# Autodesk Inventor assembly: Assembly1
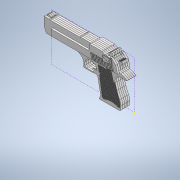
[picture p0: Inventor's stored thumbnail of the model, 180x180]
Saved by Autodesk Inventor 2022 (Build 260153000, 153)
## iProperties
Created: 2022-05-17
Part Number: Assembly1
Document SubType Name: Weldment
Designer: joshn
Weld Material: Welded Aluminum-6061
Author: joshn
## Documents named in this file (9)
- D:\Joshwin Emmanuel\Fab_accad\git_hub\Fab_Work\Wild card\Assembly\Assembly1.iam
- D:\Joshwin Emmanuel\Fab_accad\git_hub\Fab_Work\Wild card\sheetmettaal.ipt
- D:\Joshwin Emmanuel\Fab_accad\git_hub\Fab_Work\Wild card\sheetmettaal_2.ipt
- D:\Joshwin Emmanuel\Fab_accad\git_hub\Fab_Work\Wild card\sheetmettaal_3.ipt
- D:\Joshwin Emmanuel\Fab_accad\git_hub\Fab_Work\Wild card\slider.ipt
- D:\Joshwin Emmanuel\Fab_accad\git_hub\Fab_Work\Wild card\TRIGGER_1.ipt
- D:\Joshwin Emmanuel\Fab_accad\git_hub\Fab_Work\Wild card\TRIGGER_2.ipt
- D:\Joshwin Emmanuel\Fab_accad\git_hub\Fab_Work\Wild card\inner slider.ipt
- D:\Joshwin Emmanuel\Fab_accad\git_hub\Fab_Work\Wild card\FINALcASEING.ipt
## Components (20 placed, 8 different names)
1. sheetmettaal:1 — Mate:1, Mate:2, Mate:3, Mate:4, Flush:1, Flush:2, Mate:7, Flush:6, Flush:12, Flush:22, Flush:32, Mate:34, Mate:35
2. sheetmettaal_2:1 — Mate:4, Flush:1, Flush:2, Flush:3
3. sheetmettaal_3:1 — Flush:3, Mate:5, Flush:4, Flush:5, Flush:8
4. sheetmettaal_2:2 — Mate:5, Flush:4, Flush:5, Mate:8, Mate:9, Mate:11, Flush:11
5. slider:1 — Mate:7, Flush:6, Flush:7, Flush:13
6. slider:2 — Mate:8, Mate:9, Flush:7, Flush:28, Flush:29
7. TRIGGER_1:1 — Flush:8, Flush:10, Mate:17, Flush:25, Flush:26
8. TRIGGER_2:1 — Mate:10, Flush:9, Mate:17, Flush:25, Flush:26
9. TRIGGER_1:2 — Mate:10, Flush:9, Flush:10
10. sheetmettaal:2 — Mate:11, Flush:11, Flush:12, Mate:16, Mate:18
11. inner slider:1 — Flush:13, Flush:14, Mate:12, Flush:15, Mate:13, Flush:17
12. inner slider:2 — Flush:18, Flush:19, Mate:14, Mate:15, Flush:21
13. inner slider:3 — Flush:14, Mate:12, Flush:15, Flush:16
14. inner slider:4 — Flush:16, Mate:13, Flush:17, Mate:15, Flush:20, Flush:21
15. inner slider:5 — Flush:18, Flush:19, Mate:14, Flush:20, Flush:23, Flush:27
16. FINALcASEING:1 — Flush:22, Flush:24
17. FINALcASEING:2 — Mate:16, Flush:23, Flush:24, Flush:27
18. slider:3 — Mate:18, Flush:28, Flush:29
19. slider:4 — Mate:35
20. slider:5 — Flush:32, Mate:34
## Relationships (51: Flush 32, Mate 19)
- Mate:1: sheetmettaal:1
- Mate:2: sheetmettaal:1
- Mate:3: sheetmettaal:1
- Mate:4: sheetmettaal:1 ↔ sheetmettaal_2:1
- Flush:1: sheetmettaal:1 ↔ sheetmettaal_2:1
- Flush:2: sheetmettaal:1 ↔ sheetmettaal_2:1
- Flush:3: sheetmettaal_2:1 ↔ sheetmettaal_3:1
- Mate:5: sheetmettaal_3:1 ↔ sheetmettaal_2:2
- Flush:4: sheetmettaal_3:1 ↔ sheetmettaal_2:2
- Flush:5: sheetmettaal_3:1 ↔ sheetmettaal_2:2
- Mate:7: sheetmettaal:1 ↔ slider:1
- Flush:6: sheetmettaal:1 ↔ slider:1
- Mate:8: sheetmettaal_2:2 ↔ slider:2
- Mate:9: sheetmettaal_2:2 ↔ slider:2
- Flush:7: slider:1 ↔ slider:2
- Flush:8: sheetmettaal_3:1 ↔ TRIGGER_1:1
- Mate:10: TRIGGER_2:1 ↔ TRIGGER_1:2
- Flush:9: TRIGGER_2:1 ↔ TRIGGER_1:2
- Flush:10: TRIGGER_1:1 ↔ TRIGGER_1:2
- Mate:11: sheetmettaal_2:2 ↔ sheetmettaal:2
- Flush:11: sheetmettaal_2:2 ↔ sheetmettaal:2
- Flush:12: sheetmettaal:1 ↔ sheetmettaal:2
- Flush:13: slider:1 ↔ inner slider:1
- Flush:14: inner slider:1 ↔ inner slider:3
- Mate:12: inner slider:1 ↔ inner slider:3
- Flush:15: inner slider:1 ↔ inner slider:3
- Flush:16: inner slider:3 ↔ inner slider:4
- Mate:13: inner slider:1 ↔ inner slider:4
- Flush:17: inner slider:1 ↔ inner slider:4
- Flush:18: inner slider:2 ↔ inner slider:5
- Flush:19: inner slider:2 ↔ inner slider:5
- Mate:14: inner slider:2 ↔ inner slider:5
- Mate:15: inner slider:2 ↔ inner slider:4
- Flush:20: inner slider:4 ↔ inner slider:5
- Flush:21: inner slider:2 ↔ inner slider:4
- Flush:22: sheetmettaal:1 ↔ FINALcASEING:1
- Mate:16: sheetmettaal:2 ↔ FINALcASEING:2
- Flush:23: inner slider:5 ↔ FINALcASEING:2
- Flush:24: FINALcASEING:1 ↔ FINALcASEING:2
- Mate:17: TRIGGER_1:1 ↔ TRIGGER_2:1
- Flush:25: TRIGGER_1:1 ↔ TRIGGER_2:1
- Flush:26: TRIGGER_1:1 ↔ TRIGGER_2:1
- Flush:27: inner slider:5 ↔ FINALcASEING:2
- Mate:18: sheetmettaal:2 ↔ slider:3
- Flush:28: slider:2 ↔ slider:3
- Flush:29: slider:2 ↔ slider:3
- [Flush]: slider:4 ↔ slider:5
- [Flush]: slider:4 ↔ slider:5
- Flush:32: sheetmettaal:1 ↔ slider:5
- Mate:34: sheetmettaal:1 ↔ slider:5
- Mate:35: sheetmettaal:1 ↔ slider:4
## Named parameters: d53_d51 = 0 mm, d54_d52 = 0 mm
